# Autodesk Inventor assembly: AQS Assembly Test
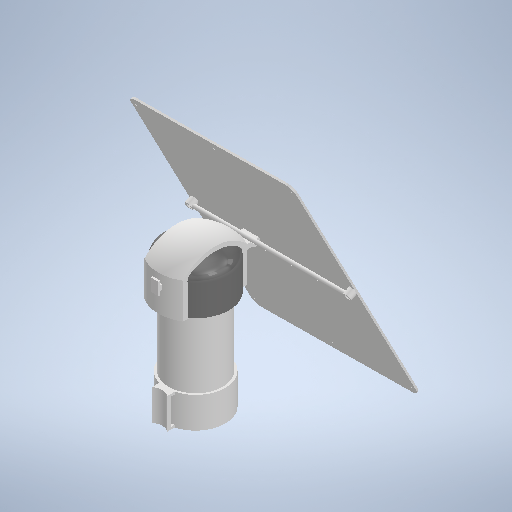
[picture p0: Inventor's stored thumbnail of the model, 512x512]
Saved by Autodesk Inventor 2025 (Build 290162010, 162A)
## iProperties
Created: 2024-07-03
Part Number: AQS Assembly Test
Document SubType Name: Assembly
Designer: vncnt
Author: vncnt
## Documents named in this file (11)
- C:\Users\vncnt\Documents\GitHub\Air-Quality-Sensor\M_CAD-Inventor\AQS Assembly Test.iam
- C:\Users\vncnt\Documents\GitHub\Air-Quality-Sensor\M_CAD-Inventor\PVC.ipt
- C:\Users\vncnt\Documents\GitHub\Air-Quality-Sensor\M_CAD-Inventor\CSL_AQS_V1_spin3.iam
- C:\Users\vncnt\Documents\GitHub\Air-Quality-Sensor\M_CAD-Inventor\AQS_Mount.ipt
- C:\Users\vncnt\Documents\GitHub\Air-Quality-Sensor\M_CAD-Inventor\SEN5X_Mount.ipt
- C:\Users\vncnt\Documents\GitHub\Air-Quality-Sensor\M_CAD-Inventor\Sensirion_STEP_SEN5x\Sensirion_STEP_SEN5x.ipt
- C:\Users\vncnt\Documents\GitHub\Air-Quality-Sensor\M_CAD-Inventor\3in End Cap\3in End Cap.ipt
- C:\Users\vncnt\Documents\GitHub\Air-Quality-Sensor\M_CAD-Inventor\Solar_Panel_Mount.ipt
- C:\Users\vncnt\Documents\GitHub\Air-Quality-Sensor\M_CAD-Inventor\Solar_Panel_Bar.ipt
- C:\Users\vncnt\Documents\GitHub\Air-Quality-Sensor\M_CAD-Inventor\Solar_Panel.ipt
- C:\Users\vncnt\Documents\GitHub\Air-Quality-Sensor\M_CAD-Inventor\Mount.ipt
## Components (10 placed, 10 different names)
1. PVC:1 — Flush:1, Mate:11, Flush:2, Mate:12, Mate:13, Flush:3, Flush:4, Flush:7, Flush:8, Flush:9, Mate:17, Flush:11, Flush:12
2. SEN5X_Mount:1 — Mate:2, Mate:3, Mate:4, Mate:5, Mate:6, Mate:7
3. Sensirion_STEP_SEN5x:1 — Mate:4, Mate:6, Mate:7
4. CSL_AQS_V1_spin3:1 [sub-assembly] — Mate:2, Mate:3, Mate:5, Mate:14
5. 3in End Cap:1 — Flush:1, Mate:11, Flush:2, Flush:5
6. AQS_Mount:1 — Mate:12, Mate:13, Mate:14
7. Solar_Panel_Mount:1 — Flush:3, Flush:4, Flush:5, Mate:15
8. Solar_Panel_Bar:1 — Mate:15, Mate:16, Angle:1
9. Solar_Panel:1 — Mate:16, Angle:1
10. Mount:1 — Mate:17, Flush:11, Flush:12
## Relationships (24: Mate 13, Flush 10, Angle 1)
- Mate:2: SEN5X_Mount:1 ↔ CSL_AQS_V1_spin3:1
- Mate:3: SEN5X_Mount:1 ↔ CSL_AQS_V1_spin3:1
- Mate:4: SEN5X_Mount:1 ↔ Sensirion_STEP_SEN5x:1
- Mate:5: SEN5X_Mount:1 ↔ CSL_AQS_V1_spin3:1
- Mate:6: SEN5X_Mount:1 ↔ Sensirion_STEP_SEN5x:1
- Mate:7: SEN5X_Mount:1 ↔ Sensirion_STEP_SEN5x:1
- Flush:1: PVC:1 ↔ 3in End Cap:1
- Mate:11: PVC:1 ↔ 3in End Cap:1
- Flush:2: PVC:1 ↔ 3in End Cap:1
- Mate:12: PVC:1 ↔ AQS_Mount:1
- Mate:13: PVC:1 ↔ AQS_Mount:1
- Mate:14: CSL_AQS_V1_spin3:1 ↔ AQS_Mount:1
- Flush:3: PVC:1 ↔ Solar_Panel_Mount:1
- Flush:4: PVC:1 ↔ Solar_Panel_Mount:1
- Flush:5 (-45.339 mm): 3in End Cap:1 ↔ Solar_Panel_Mount:1
- Flush:7: PVC:1
- Flush:8: PVC:1
- Flush:9: PVC:1
- Mate:15: Solar_Panel_Mount:1 ↔ Solar_Panel_Bar:1
- Mate:16: Solar_Panel_Bar:1 ↔ Solar_Panel:1
- Angle:1 (0 deg): Solar_Panel_Bar:1 ↔ Solar_Panel:1
- Mate:17: PVC:1 ↔ Mount:1
- Flush:11: PVC:1 ↔ Mount:1
- Flush:12 (2.0066 mm): PVC:1 ↔ Mount:1
